# Autodesk Inventor assembly: Many Wrenches
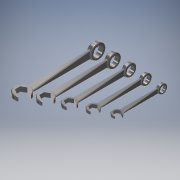
[picture p0: Inventor's stored thumbnail of the model, 180x180]
Saved by Autodesk Inventor 2018 (Build 220112000, 112)
## iProperties
Created: 2017-11-02
Part Number: Many Wrenches
Document SubType Name: Assembly
Designer: kurtis
Author: kurtis
## Documents named in this file (7)
- D:\Users\kurti\Git-Home\CAD\GE101\MA8\Many Wrenches.iam
- D:\Users\kurti\Git-Home\CAD\GE101\MA8\Wrench\Wrench-01.ipt
- D:\Users\kurti\Git-Home\CAD\GE101\MA8\Wrench.ipt
- D:\Users\kurti\Git-Home\CAD\GE101\MA8\Wrench\Wrench-02.ipt
- D:\Users\kurti\Git-Home\CAD\GE101\MA8\Wrench\Wrench-03.ipt
- D:\Users\kurti\Git-Home\CAD\GE101\MA8\Wrench\Wrench-04.ipt
- D:\Users\kurti\Git-Home\CAD\GE101\MA8\Wrench\Wrench-05.ipt
## Components (5 placed, 5 different names)
1. Wrench-01:2 — Rotational:1, Planar:4, Mate:1
2. Wrench-02:3 — Rotational:1, Rotational:2, Planar:1, Planar:4
3. Wrench-03:4 — Rotational:2, Rotational:3, Planar:1, Planar:2
4. Wrench-04:5 — Rotational:3, Rotational:4, Planar:2, Planar:3
5. Wrench-05:6 — Rotational:4, Planar:3
## Relationships (9: RevoluteJoint 4, PlanarJoint 4, Mate 1)
- Rotational:1 [RevoluteJoint] (35 mm): Wrench-01:2 ↔ Wrench-02:3
- Rotational:2 [RevoluteJoint] (35 mm): Wrench-02:3 ↔ Wrench-03:4
- Rotational:3 [RevoluteJoint] (35 mm): Wrench-03:4 ↔ Wrench-04:5
- Rotational:4 [RevoluteJoint] (35 mm): Wrench-04:5 ↔ Wrench-05:6
- Planar:1: Wrench-02:3 ↔ Wrench-03:4
- Planar:2: Wrench-03:4 ↔ Wrench-04:5
- Planar:3: Wrench-04:5 ↔ Wrench-05:6
- Planar:4: Wrench-01:2 ↔ Wrench-02:3
- Mate:1: Wrench-01:2
## Named parameters: Dist = 35 mm
